# Autodesk Inventor assembly: case_assembly
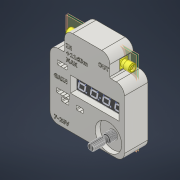
[picture p0: Inventor's stored thumbnail of the model, 180x180]
Saved by Autodesk Inventor 2022 (Build 260153000, 153)
## iProperties
Created: 2021-12-11
Part Number: case_assembly
Document SubType Name: Assembly
Designer: nebst
Author: nebst
## Documents named in this file (4)
- D:\Documents\Git_Local\rf-vga\pcb\case\case_assembly.iam
- D:\Documents\Git_Local\rf-vga\pcb\case\rf-vga.iam
- D:\Documents\Git_Local\rf-vga\pcb\case\shell.ipt
- D:\Documents\Git_Local\rf-vga\pcb\case\sliding cover.ipt
## Components (3 placed, 3 different names)
1. rf-vga:1 [sub-assembly] — Flush:1, Flush:2, Flush:3
2. shell:1 — Flush:1, Flush:2, Flush:3, Flush:4
3. sliding cover:1 — Flush:4
## Relationships (4: Flush 4)
- Flush:1: rf-vga:1 ↔ shell:1
- Flush:2: rf-vga:1 ↔ shell:1
- Flush:3: rf-vga:1 ↔ shell:1
- Flush:4: shell:1 ↔ sliding cover:1
